# Autodesk Inventor assembly: ASY MSC 100 CONE
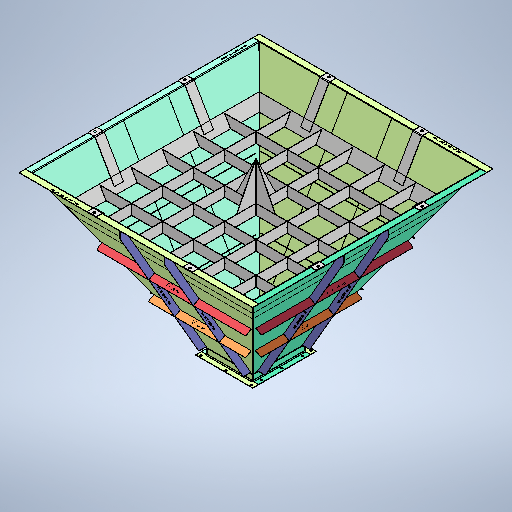
[picture p0: Inventor's stored thumbnail of the model, 512x512]
Saved by Autodesk Inventor 2025.1 (Build 291241020, 241B)
## iProperties
Created: 2024-05-19
Part Number: ASY MSC 100 CONE
Document SubType Name: Assembly
Designer: admin
Mass: 214616 g
Surface Area: 182315 cm^2
Volume: 26827 cm^3
Density: 8 g/cm^3
Stock Number: ASY МОО 100 конус
Author: admin
## Documents named in this file (19)
- C:\Users\user\YandexDisk-badmisterfox\домашниий пк\Inventor\NDM-VOS_powder_hopper\Workspaces\Workspace\Cone\ASY MSC 100 cone.iam
- C:\Users\user\YandexDisk-badmisterfox\домашниий пк\Inventor\NDM-VOS_powder_hopper\Workspaces\Workspace\Cone\MSC 114 cone IN right board.ipt
- C:\Users\user\YandexDisk-badmisterfox\домашниий пк\Inventor\NDM-VOS_powder_hopper\Workspaces\Workspace\Cone\MSC 113 cone IN left board.ipt
- C:\Users\user\YandexDisk-badmisterfox\домашниий пк\Inventor\NDM-VOS_powder_hopper\Workspaces\Workspace\Cone\MSC 112 cone IN back.ipt
- C:\Users\user\YandexDisk-badmisterfox\домашниий пк\Inventor\NDM-VOS_powder_hopper\Workspaces\Workspace\Cone\MSC DIM 001 cone sketch.ipt
- C:\Users\user\YandexDisk-badmisterfox\домашниий пк\Inventor\NDM-VOS_powder_hopper\Workspaces\Workspace\Cone\MSC 115 cone IN bow.ipt
- C:\Users\user\YandexDisk-badmisterfox\домашниий пк\Inventor\NDM-VOS_powder_hopper\Workspaces\Workspace\Cone\MSC 110 stringer cone.ipt
- C:\Users\user\YandexDisk-badmisterfox\домашниий пк\Inventor\NDM-VOS_powder_hopper\Workspaces\Workspace\Cone\MSC 106 rib cone.ipt
- C:\Users\user\YandexDisk-badmisterfox\домашниий пк\Inventor\NDM-VOS_powder_hopper\Workspaces\Workspace\Cone\MSC 107 rib cone.ipt
- C:\Users\user\YandexDisk-badmisterfox\домашниий пк\Inventor\NDM-VOS_powder_hopper\Workspaces\Workspace\Cone\MSC 108 rib cone.ipt
- C:\Users\user\YandexDisk-badmisterfox\домашниий пк\Inventor\NDM-VOS_powder_hopper\Workspaces\Workspace\Cone\MSC 109 rib cone.ipt
- C:\Users\user\YandexDisk-badmisterfox\домашниий пк\Inventor\NDM-VOS_powder_hopper\NDM-VOS dummy2.ipt
- C:\Users\user\YandexDisk-badmisterfox\домашниий пк\Inventor\NDM-VOS_powder_hopper\Workspaces\Workspace\Cone\MSC 201 GRID.ipt
- C:\Users\user\YandexDisk-badmisterfox\домашниий пк\Inventor\NDM-VOS_powder_hopper\Workspaces\Workspace\Cone\MSC 202 GRID CORNER.ipt
- C:\Users\user\YandexDisk-badmisterfox\домашниий пк\Inventor\NDM-VOS_powder_hopper\Workspaces\Workspace\Cone\MSC 206 GRID_CPY.ipt
- C:\Users\user\YandexDisk-badmisterfox\домашниий пк\Inventor\NDM-VOS_powder_hopper\Workspaces\Workspace\Cone\MSC 203 GRID.ipt
- C:\Users\user\YandexDisk-badmisterfox\домашниий пк\Inventor\NDM-VOS_powder_hopper\Workspaces\Workspace\Cone\MSC 204 GRID.ipt
- C:\Users\user\YandexDisk-badmisterfox\домашниий пк\Inventor\NDM-VOS_powder_hopper\Workspaces\Workspace\Cone\MSC 205 CONE BLADE.ipt
- C:\Users\user\YandexDisk-badmisterfox\домашниий пк\Inventor\NDM-VOS_powder_hopper\Workspaces\Workspace\Cone\MSC 207 CONE BLADE.ipt
## Components (47 placed, 24 different names)
1. NDM-VOS dummy2:1 — Mate:73, Mate:74, Flush:19
2. MSC DIM 001 CONE SKETCH:1 — Flush:8, Flush:9, Mate:1
3. MSC 112 CONE IN BACK:1 — Flush:6, Flush:10, Mate:2
4. MSC 114 CONE IN RIGHT BOARD:1 — Flush:13, Flush:15, Flush:18, Mate:79, Mate:81, Mate:90, Mate:93
5. MSC 113 CONE IN LEFT BOARD:1 — Mate:4, Flush:14, Mate:5, Mate:98, Mate:99
6. MSC 115 CONE IN BOW:1 — Mate:6, Flush:16, Flush:17, Mate:88, Mate:94, Mate:95
7. MSC 115 cone IN bow:2 — Mate:75, Flush:20, Flush:21, Mate:76, Mate:78, Mate:102, Mate:103
8. MSC 202 GRID CORNER:1 — Mate:90, Mate:91
9. MSC 206 GRID_CPY:2 — Rigid:15, Mate:88, Mate:96, Mate:97
10. MSC 206 GRID_CPY:4 — Rigid:17, Mate:104, Mate:105
11. MSC 204 GRID:1 — Rigid:20, Mate:91, Mate:92
12. MSC 204 GRID:2 — Rigid:21, Mate:100, Mate:101
13. MSC 205 CONE BLADE:1 — Rigid:23, Rigid:24
14. MSC 207 CONE BLADE:1 — Rigid:23
15. MSC 202 GRID CORNER:2 — Mate:92, Mate:93
16. MSC 202 GRID CORNER:3 — Mate:102, Mate:105
17. MSC 202 GRID CORNER:4 — Mate:103, Mate:104
18. MSC 202 GRID CORNER:5 — Mate:98, Mate:100
19. MSC 202 GRID CORNER:6 — Mate:99, Mate:101
20. MSC 202 GRID CORNER:7 — Mate:95, Mate:96
21. MSC 202 GRID CORNER:8 — Mate:94, Mate:97
22. MSC 106 RIB CONE:1 — Rigid:7, Rigid:8, Mate:77
23. MSC 109 RIB CONE:1 — Rigid:6
24. MSC 110 STRINGER CONE:4 — Rigid:4, Rigid:6, Mate:79, Mate:81
25. MSC 108 RIB CONE:1 — Rigid:4, Rigid:5, Mate:80
26. MSC 110 STRINGER CONE:3 — Rigid:5
27. MSC 110 STRINGER CONE:2 — Rigid:8, Rigid:9
28. MSC 107 RIB CONE:1 — Rigid:9
29. MSC 110 STRINGER CONE:1 — Rigid:7, Mate:76, Mate:78
30. MSC 106 rib cone:2
31. MSC 109 rib cone:2
32. MSC 110 stringer cone:6
33. MSC 108 rib cone:2
34. MSC 110 stringer cone:7
35. MSC 110 stringer cone:8
36. MSC 107 rib cone:2
37. MSC 110 stringer cone:9
38. MSC 203 GRID:1 — Mate:89, Flush:22, Flush:23, Rigid:20, Rigid:21, Rigid:24
39. MSC 203 GRID:2
40. MSC 203 GRID:3
41. MSC 203 GRID:4
42. MSC 203 GRID:5
43. MSC 201 GRID:2 — Mate:84, Mate:86, Rigid:15, Rigid:17, Flush:22
44. MSC 201 GRID:3
45. MSC 201 GRID:4
46. MSC 201 GRID:5
47. MSC 201 GRID:6
## Component patterns: (2 elements, first: MSC 106 RIB CONE:1 + MSC 109 RIB CONE:1 + MSC 110 STRINGER CONE:4 + MSC 108 RIB CONE:1 + MSC 110 STRINGER CONE:3 + MSC 110 STRINGER CONE:2 + MSC 107 RIB CONE:1 + MSC 110 STRINGER CONE:1), (5 elements, first: MSC 203 GRID:1), (5 elements, first: MSC 201 GRID:2)
## Relationships (61: Mate 34, Flush 15, WeldJoint 12)
- Flush:6: MSC 112 CONE IN BACK:1
- Flush:8: MSC DIM 001 CONE SKETCH:1
- Flush:9: MSC DIM 001 CONE SKETCH:1
- Mate:1: MSC DIM 001 CONE SKETCH:1
- Flush:10: MSC 112 CONE IN BACK:1
- Mate:2: MSC 112 CONE IN BACK:1
- Flush:13: MSC 114 CONE IN RIGHT BOARD:1
- Mate:4: MSC 113 CONE IN LEFT BOARD:1
- Flush:14: MSC 113 CONE IN LEFT BOARD:1
- Mate:5: MSC 113 CONE IN LEFT BOARD:1
- Flush:15: MSC 114 CONE IN RIGHT BOARD:1
- Mate:6: MSC 115 CONE IN BOW:1
- Flush:16: MSC 115 CONE IN BOW:1
- Flush:17: MSC 115 CONE IN BOW:1
- Rigid:4 [WeldJoint] (2 mm): MSC 110 STRINGER CONE:4 ↔ MSC 108 RIB CONE:1
- Rigid:5 [WeldJoint] (2 mm): MSC 108 RIB CONE:1 ↔ MSC 110 STRINGER CONE:3
- Rigid:6 [WeldJoint] (2 mm): MSC 109 RIB CONE:1 ↔ MSC 110 STRINGER CONE:4
- Rigid:7 [WeldJoint] (2 mm): MSC 106 RIB CONE:1 ↔ MSC 110 STRINGER CONE:1
- Rigid:8 [WeldJoint] (2 mm): MSC 106 RIB CONE:1 ↔ MSC 110 STRINGER CONE:2
- Rigid:9 [WeldJoint] (2 mm): MSC 110 STRINGER CONE:2 ↔ MSC 107 RIB CONE:1
- Flush:18: MSC 114 CONE IN RIGHT BOARD:1
- Mate:73: NDM-VOS dummy2:1
- Mate:74: NDM-VOS dummy2:1
- Flush:19: NDM-VOS dummy2:1
- Mate:75: MSC 115 cone IN bow:2
- Flush:20: MSC 115 cone IN bow:2
- Flush:21: MSC 115 cone IN bow:2
- Mate:76: MSC 115 cone IN bow:2 ↔ MSC 110 STRINGER CONE:1
- Mate:77: MSC 106 RIB CONE:1
- Mate:78 (2 mm): MSC 115 cone IN bow:2 ↔ MSC 110 STRINGER CONE:1
- Mate:79: MSC 114 CONE IN RIGHT BOARD:1 ↔ MSC 110 STRINGER CONE:4
- Mate:80: MSC 108 RIB CONE:1
- Mate:81 (4 mm): MSC 114 CONE IN RIGHT BOARD:1 ↔ MSC 110 STRINGER CONE:4
- Mate:84: MSC 201 GRID:2
- Mate:86: MSC 201 GRID:2
- Rigid:15 [WeldJoint]: MSC 206 GRID_CPY:2 ↔ MSC 201 GRID:2
- Rigid:17 [WeldJoint]: MSC 206 GRID_CPY:4 ↔ MSC 201 GRID:2
- Mate:88: MSC 115 CONE IN BOW:1 ↔ MSC 206 GRID_CPY:2
- Mate:89: MSC 203 GRID:1
- Flush:22: MSC 203 GRID:1 ↔ MSC 201 GRID:2
- Flush:23: MSC 203 GRID:1
- Rigid:20 [WeldJoint]: MSC 204 GRID:1 ↔ MSC 203 GRID:1
- Rigid:21 [WeldJoint]: MSC 204 GRID:2 ↔ MSC 203 GRID:1
- Rigid:23 [WeldJoint] (2 mm): MSC 205 CONE BLADE:1 ↔ MSC 207 CONE BLADE:1
- Rigid:24 [WeldJoint]: MSC 205 CONE BLADE:1 ↔ MSC 203 GRID:1
- Mate:90: MSC 114 CONE IN RIGHT BOARD:1 ↔ MSC 202 GRID CORNER:1
- Mate:91: MSC 202 GRID CORNER:1 ↔ MSC 204 GRID:1
- Mate:92: MSC 204 GRID:1 ↔ MSC 202 GRID CORNER:2
- Mate:93: MSC 114 CONE IN RIGHT BOARD:1 ↔ MSC 202 GRID CORNER:2
- Mate:94: MSC 115 CONE IN BOW:1 ↔ MSC 202 GRID CORNER:8
- Mate:95: MSC 115 CONE IN BOW:1 ↔ MSC 202 GRID CORNER:7
- Mate:96: MSC 206 GRID_CPY:2 ↔ MSC 202 GRID CORNER:7
- Mate:97: MSC 206 GRID_CPY:2 ↔ MSC 202 GRID CORNER:8
- Mate:98: MSC 113 CONE IN LEFT BOARD:1 ↔ MSC 202 GRID CORNER:5
- Mate:99: MSC 113 CONE IN LEFT BOARD:1 ↔ MSC 202 GRID CORNER:6
- Mate:100: MSC 204 GRID:2 ↔ MSC 202 GRID CORNER:5
- Mate:101: MSC 204 GRID:2 ↔ MSC 202 GRID CORNER:6
- Mate:102: MSC 115 cone IN bow:2 ↔ MSC 202 GRID CORNER:3
- Mate:103: MSC 115 cone IN bow:2 ↔ MSC 202 GRID CORNER:4
- Mate:104: MSC 206 GRID_CPY:4 ↔ MSC 202 GRID CORNER:4
- Mate:105: MSC 206 GRID_CPY:4 ↔ MSC 202 GRID CORNER:3
## Named parameters: Конус_Базовая_Высота = 1170 mm, Конус_отступ_от_пола = 0 mm
